# Autodesk Inventor assembly: AssiemeGiusto
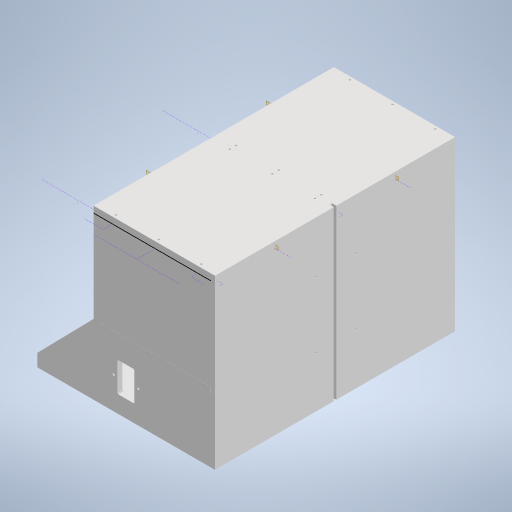
[picture p0: Inventor's stored thumbnail of the model, 512x512]
Saved by Autodesk Inventor 2024.2 (Build 282272000, 272)
## iProperties
Created: 2025-07-13
Part Number: AssiemeGiusto
Document SubType Name: Assembly
Designer: zagom
Author: zagom
## Documents named in this file (14)
- C:\Users\zagom\Desktop\nuovo assieme\AssiemeGiusto.iam
- C:\Users\zagom\Desktop\nuovo assieme\Base1.ipt
- C:\Users\zagom\Desktop\nuovo assieme\Base2.ipt
- C:\Users\zagom\Desktop\nuovo assieme\Coperchi1.ipt
- C:\Users\zagom\Desktop\nuovo assieme\Coperchio2.ipt
- C:\Users\zagom\Desktop\nuovo assieme\Nextion1.ipt
- C:\Users\zagom\Desktop\nuovo assieme\Nextion2.ipt
- C:\Users\zagom\Desktop\nuovo assieme\PortaCassetto1.ipt
- C:\Users\zagom\Desktop\nuovo assieme\Parte_frontale.ipt
- C:\Users\zagom\Desktop\nuovo assieme\ParteCassetto.ipt
- C:\Users\zagom\Desktop\nuovo assieme\PiattoBilancia.ipt
- C:\Users\zagom\Desktop\nuovo assieme\Coperchio.ipt
- C:\Users\zagom\Desktop\nuovo assieme\Porticina11.ipt
- C:\Users\zagom\Desktop\nuovo assieme\Porticina22.ipt
## Components (20 placed, 13 different names)
1. Base1:1 — Rigido:1, Rigido:3, Rigido:15
2. Base2:1 — Rigido:1, Rigido:5, Rigido:14
3. Coperchi1:1 — Rigido:2
4. Coperchio2:1 — Rigido:2, Rigido:3
5. Nextion1:1 — Rigido:4, Rigido:6
6. Nextion2:1 — Rigido:4, Rigido:5, Rigido:7
7. PortaCassetto1:1 — Rigido:6, Rigido:9, Rotazionale:3
8. PortaCassetto1:2 — Rigido:7, Rigido:8, Rotazionale:4
9. Parte_frontale:1 — Rigido:8, Rotazionale:2
10. Parte_frontale:2 — Rigido:9, Rotazionale:1
11. ParteCassetto:1 — Rotazionale:1, Rigido:11
12. ParteCassetto:2 — Rotazionale:2, Rigido:10
13. PiattoBilancia:1 — Rigido:10
14. PiattoBilancia:2 — Rigido:11
15. Coperchio:1 — Rotazionale:3
16. Coperchio:2 — Rotazionale:4
17. Porticina11:1 — Rigido:12
18. Porticina11:2 — Rigido:13, Rigido:15
19. Porticina22:1 — Rigido:12, Rigido:14
20. Porticina22:2 — Rigido:13
## Relationships (19: WeldJoint 15, RevoluteJoint 4)
- Rigido:1 [WeldJoint]: Base1:1 ↔ Base2:1
- Rigido:2 [WeldJoint]: Coperchi1:1 ↔ Coperchio2:1
- Rigido:3 [WeldJoint]: Base1:1 ↔ Coperchio2:1
- Rigido:4 [WeldJoint]: Nextion1:1 ↔ Nextion2:1
- Rigido:5 [WeldJoint]: Base2:1 ↔ Nextion2:1
- Rigido:6 [WeldJoint]: Nextion1:1 ↔ PortaCassetto1:1
- Rigido:7 [WeldJoint]: Nextion2:1 ↔ PortaCassetto1:2
- Rigido:8 [WeldJoint]: PortaCassetto1:2 ↔ Parte_frontale:1
- Rigido:9 [WeldJoint]: PortaCassetto1:1 ↔ Parte_frontale:2
- Rotazionale:1 [RevoluteJoint]: Parte_frontale:2 ↔ ParteCassetto:1
- Rotazionale:2 [RevoluteJoint]: Parte_frontale:1 ↔ ParteCassetto:2
- Rigido:10 [WeldJoint]: ParteCassetto:2 ↔ PiattoBilancia:1
- Rigido:11 [WeldJoint]: ParteCassetto:1 ↔ PiattoBilancia:2
- Rotazionale:3 [RevoluteJoint]: PortaCassetto1:1 ↔ Coperchio:1
- Rotazionale:4 [RevoluteJoint]: PortaCassetto1:2 ↔ Coperchio:2
- Rigido:12 [WeldJoint]: Porticina11:1 ↔ Porticina22:1
- Rigido:13 [WeldJoint]: Porticina11:2 ↔ Porticina22:2
- Rigido:14 [WeldJoint]: Base2:1 ↔ Porticina22:1
- Rigido:15 [WeldJoint]: Base1:1 ↔ Porticina11:2
